# Autodesk Inventor assembly: treasureChest
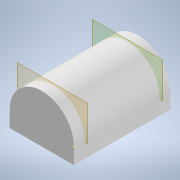
[picture p0: Inventor's stored thumbnail of the model, 180x180]
Saved by Autodesk Inventor 2020.3 (Build 243373000, 373)
## iProperties
Created: 2021-02-24
Part Number: treasureChest
Document SubType Name: Assembly
Designer: con_c_000
Author: con_c_000
## Documents named in this file (3)
- C:\Users\con_c_000\Documents\Inventor\Content Center Files\FIRST ROBOT\treasureChest.iam
- C:\Users\con_c_000\Documents\Inventor\Content Center Files\FIRST ROBOT\chestTop.ipt
- C:\Users\con_c_000\Documents\Inventor\Content Center Files\FIRST ROBOT\chestLower.ipt
## Components (2 placed, 2 different names)
1. chestTop:1 — Rotational:1
2. chestLower:1 — Rotational:1
## Relationships (1: RevoluteJoint 1)
- Rotational:1 [RevoluteJoint]: chestTop:1 ↔ chestLower:1
